# Autodesk Inventor assembly: ASY GBK короткая стенка
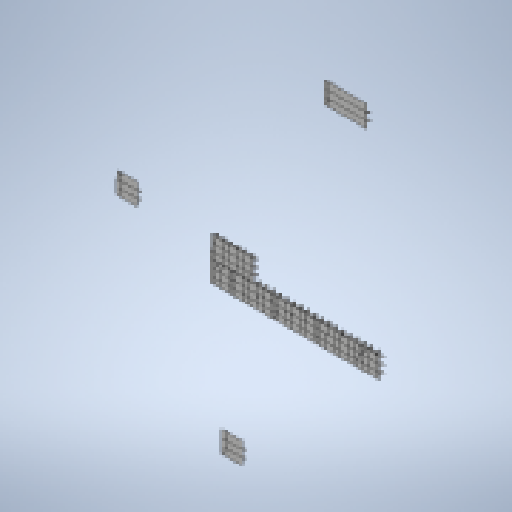
[picture p0: Inventor's stored thumbnail of the model, 512x512]
Saved by Autodesk Inventor 2026 (Build 300175000, 175)
## iProperties
Created: 2026-05-24
Part Number: ASY GBK короткая стенка
Document SubType Name: Assembly
Designer: pokla
Author: pokla
## Documents named in this file (8)
- C:\Users\pokla\Documents\Inventor\GBK-Gubkinskiy\ASY GBK короткая стенка.iam
- C:\Users\pokla\Documents\Inventor\GBK-Gubkinskiy\ASY GBK 2110 short wall shield 1.iam
- C:\Users\pokla\Documents\Inventor\GBK-Gubkinskiy\ASY GBK 2120 short wall shield 2.iam
- C:\Users\pokla\Documents\Inventor\GBK-Gubkinskiy\ASY GBK 2130 short wall shield 3.iam
- C:\Users\pokla\Documents\Inventor\GBK-Gubkinskiy\ASY GBK 2210 short wall shield 4.iam
- C:\Users\pokla\Documents\Inventor\GBK-Gubkinskiy\ASY GBK 2310 short wall shield 7.iam
- C:\Users\pokla\Documents\Inventor\GBK-Gubkinskiy\ASY GBK 2320 short wall shield 8.iam
- C:\Users\pokla\Documents\Inventor\GBK-Gubkinskiy\ASY GBK 2330 short wall shield 9.iam
## Components (9 placed, 8 different names)
1. ASY GBK 2110 short wall shield 1.iam:1 [sub-assembly] — Жесткий:1, Жесткий:5
2. ASY GBK 2120 short wall shield 2.iam:1 [sub-assembly] — Жесткий:1, Жесткий:2
3. ASY GBK 2130 short wall shield 3.iam:1 [sub-assembly] — Жесткий:4
4. ASY GBK 2210 short wall shield 4.iam:1 [sub-assembly] — Жесткий:5
5. ASY GBK 2310 short wall shield 5.iam:1 [sub-assembly]
6. ASY GBK 2320 short wall shield 6.iam:1 [sub-assembly]
7. ASY GBK 2330 short wall shield 7.iam:1 [sub-assembly]
8. ASY GBK 2120 short wall shield 2:2 [sub-assembly] — Жесткий:2, Жесткий:3
9. ASY GBK 2120 short wall shield 2:3 [sub-assembly] — Жесткий:3, Жесткий:4
## Relationships (5: WeldJoint 5)
- Жесткий:1 [WeldJoint]: ASY GBK 2110 short wall shield 1.iam:1 ↔ ASY GBK 2120 short wall shield 2.iam:1
- Жесткий:2 [WeldJoint]: ASY GBK 2120 short wall shield 2.iam:1 ↔ ASY GBK 2120 short wall shield 2:2
- Жесткий:3 [WeldJoint]: ASY GBK 2120 short wall shield 2:2 ↔ ASY GBK 2120 short wall shield 2:3
- Жесткий:4 [WeldJoint]: ASY GBK 2130 short wall shield 3.iam:1 ↔ ASY GBK 2120 short wall shield 2:3
- Жесткий:5 [WeldJoint]: ASY GBK 2110 short wall shield 1.iam:1 ↔ ASY GBK 2210 short wall shield 4.iam:1
